# Autodesk Inventor assembly: WristRot
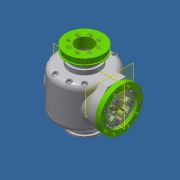
[picture p0: Inventor's stored thumbnail of the model, 180x180]
Saved by Autodesk Inventor 2016 (Build 200138000, 138)
## iProperties
Created: 2016-03-29
Part Number: WristRot
Material: Generisch
Document SubType Name: Assembly
Designer: 4ndreas
Mass: 560.727 g
Surface Area: 1571.35 cm^2
Volume: 276.943 cm^3
Density: 2.0247 g/cm^3
Parent: R5
Author: 4ndreas
## Documents named in this file (36)
- C:\Users\4ndreas\Documents\Inventor\betabots Mantis\Workspaces\Arbeitsbereich\v4\_assemblys\WristRot.iam
- C:\Users\4ndreas\Documents\Inventor\betabots Mantis\Workspaces\Arbeitsbereich\v4\_printed parts\WristRot_A.ipt
- C:\Users\4ndreas\Documents\Inventor\betabots Mantis\Workspaces\Arbeitsbereich\v4\_printed parts\WristRot_B.ipt
- C:\Users\4ndreas\Documents\Inventor\betabots Mantis\Workspaces\Arbeitsbereich\v4\_printed parts\WristRot_C.ipt
- C:\Users\4ndreas\Documents\Inventor\betabots Mantis\Workspaces\Arbeitsbereich\v4\_printed parts\WristRot_D.ipt
- C:\Users\4ndreas\Documents\Inventor\betabots Mantis\Workspaces\Arbeitsbereich\v4\_printed parts\WristRot_E.ipt
- C:\Users\4ndreas\Documents\Inventor\betabots Mantis\Workspaces\Arbeitsbereich\v4\_standard Parts\Distanzhuelse_M4x20mm.ipt
- C:\Users\4ndreas\Documents\Inventor\betabots Mantis\Libraries\Content Center Files\de-DE\DIN BEARING(1)\DIN 625 SKF - SKF 61807.ipt
- C:\Users\4ndreas\Documents\Inventor\betabots Mantis\Workspaces\Arbeitsbereich\v4\_Wrist_rev1\Wrist_rot_r1b\Konstruktions-Assistent\Stirnräder6.iam
- C:\Users\4ndreas\Documents\Inventor\betabots Mantis\Workspaces\Arbeitsbereich\v4\_standard Parts\Slipring_SNM012A-06.ipt
- C:\Users\4ndreas\Documents\Inventor\betabots Mantis\Libraries\Content Center Files\de-DE\DIN BEARING(1)\DIN 625 SKF - SKF 608.ipt
- C:\Users\4ndreas\Documents\Inventor\betabots Mantis\Workspaces\Arbeitsbereich\v4\_encoder\EncoderMagnet.ipt
- C:\Users\4ndreas\Documents\Inventor\betabots Mantis\Workspaces\Arbeitsbereich\v4\_Wrist_rev1\GripperRot.ipt
- C:\Users\4ndreas\Documents\Inventor\betabots Mantis\Libraries\Content Center Files\de-DE\DIN 125-1  A\DIN 125 - A 8,4.ipt
- C:\Users\4ndreas\Documents\Inventor\betabots Mantis\Workspaces\Arbeitsbereich\v4\_metal parts\SlipRingExtender.ipt
- C:\Users\4ndreas\Documents\Inventor\betabots Mantis\Libraries\Content Center Files\de-DE\DIN 985\DIN 985 - M6.ipt
- C:\Users\4ndreas\Documents\Inventor\betabots Mantis\Workspaces\Arbeitsbereich\v4\_Wrist_rev1\Wrist_rot_r1b\Konstruktions-Assistent\Stirnräder1.iam
- C:\Users\4ndreas\Documents\Inventor\betabots Mantis\Workspaces\Arbeitsbereich\v4\_Wrist_rev1\Wrist_rot_r1b\Konstruktions-Assistent\Welle1.iam
- C:\Users\4ndreas\Documents\Inventor\betabots Mantis\Workspaces\Arbeitsbereich\v4\_Wrist_rev1\Wrist_rot_r1b\Konstruktions-Assistent\Stirnräder3.iam
- C:\Users\4ndreas\Documents\Inventor\betabots Mantis\Workspaces\Arbeitsbereich\v4\_Wrist_rev1\Wrist_rot_r1b\Konstruktions-Assistent\Welle2.iam
- C:\Users\4ndreas\Documents\Inventor\betabots Mantis\Workspaces\Arbeitsbereich\v4\_motors\Stepper_42mm.ipt
- C:\Users\4ndreas\Documents\Inventor\betabots Mantis\Libraries\Content Center Files\de-DE\DIN 912\DIN 912 - M4 x 0,7 x 20 x 18,25.ipt
- C:\Users\4ndreas\Documents\Inventor\betabots Mantis\Libraries\Content Center Files\de-DE\DIN 7991(2)\DIN 7991 - M3x16.ipt
- C:\Users\4ndreas\Documents\Inventor\betabots Mantis\Workspaces\Arbeitsbereich\v4\_Wrist_rev1\RotGear_spacer.ipt
- C:\Users\4ndreas\Documents\Inventor\betabots Mantis\Workspaces\Arbeitsbereich\v4\_Wrist_rev1\Wrist_r1\Konstruktions-Assistent\Synchrone Riemenscheibe22.ipt
- C:\Users\4ndreas\Documents\Inventor\betabots Mantis\Libraries\Content Center Files\de-DE\DIN 7991(2)\DIN 7991 - M3x30.ipt
- C:\Users\4ndreas\Documents\Inventor\betabots Mantis\Workspaces\Arbeitsbereich\v4\_Wrist_rev1\RotGear_spacer_B.ipt
- C:\Users\4ndreas\Documents\Inventor\betabots Mantis\Workspaces\Arbeitsbereich\v4\_Wrist_rev1\WristMagnetMount.ipt
- C:\Users\4ndreas\Documents\Inventor\betabots Mantis\Libraries\Content Center Files\de-DE\DIN 7991(2)\DIN 7991 - M3x20.ipt
- C:\Users\4ndreas\Documents\Inventor\betabots Mantis\Workspaces\Arbeitsbereich\v4\_Wrist_rev1\GripperMountCover.ipt
- C:\Users\4ndreas\Documents\Inventor\betabots Mantis\Workspaces\Arbeitsbereich\v4\_encoder\encoderR1_mini.ipt
- C:\Users\4ndreas\Documents\Inventor\betabots Mantis\Libraries\Content Center Files\de-DE\DIN 625 SKF(4)\DIN 625 SKF - SKF 624-2Z.ipt
- C:\Users\4ndreas\Documents\Inventor\betabots Mantis\Libraries\Content Center Files\de-DE\DIN 125-1  A\DIN 125 - A 4,3.ipt
- C:\Users\4ndreas\Documents\Inventor\betabots Mantis\Libraries\Content Center Files\de-DE\DIN 912\DIN 912 - M3 x 0,5 x 8 x 6,75.ipt
- C:\Users\4ndreas\Documents\Inventor\betabots Mantis\Workspaces\Arbeitsbereich\v4\_encoder\encoder_neu.iam
- C:\Users\4ndreas\Documents\Inventor\betabots Mantis\Workspaces\Arbeitsbereich\v4\_Wrist_rev1\Wrist_EncoderMagnetMount.ipt
## Components (76 placed, 32 different names)
1. WristRot_A:1 — Fluchtend:1, Fluchtend:2, Fluchtend:3, Passend:1, Fluchtend:4, Passend:2, Passend:7, Passend:8, Passend:9, Passend:10, Passend:12, Passend:13, Passend:14, Passend:15, Passend:16, Passend:17, Passend:18, Passend:19, Passend:36, Passend:37, Passend:38, Passend:61, Passend:64, Passend:65, Einfügen:5, Einfügen:6, Einfügen:7, Einfügen:8, Einfügen:9, Passend:76, Passend:77, Passend:78, Passend:104, Winkel:1, Passend:115, Fluchtend:49
2. WristRot_B:1 — Passend:1, Fluchtend:4, Passend:2, Passend:3, Fluchtend:5, Passend:4, Passend:6, Fluchtend:48, Winkel:2
3. WristRot_C:1 — Passend:3, Fluchtend:5, Passend:4, Passend:5, Fluchtend:6, Passend:59
4. WristRot_D:1 — Passend:5, Passend:6, Fluchtend:6, Einfügen:1, Einfügen:2, Einfügen:3, Einfügen:4, Passend:11, Passend:79, Passend:80, Passend:81, Passend:82, Passend:83
5. WristRot_E:1 — Passend:7, Passend:8, Passend:66, Passend:67, Passend:68, Passend:69, Passend:70, Passend:71, Passend:72, Passend:73, Passend:74, Passend:75
6. Distanzhuelse_M4x20mm:1 — Passend:11, Fluchtend:7, Passend:19
7. Distanzhuelse_M4x20mm:2 — Passend:9, Fluchtend:8, Passend:17
8. Distanzhuelse_M4x20mm:3 — Passend:10, Fluchtend:7, Fluchtend:8, Fluchtend:9, Passend:18
9. Distanzhuelse_M4x20mm:4 — Passend:13, Fluchtend:10, Passend:14, Passend:15
10. Distanzhuelse_M4x20mm:5 — Passend:12, Fluchtend:9, Fluchtend:10, Passend:16
11. DIN 625 SKF SKF 61807:1 — Passend:38
12. Stirnräder:1 [sub-assembly] — Passend:45, Drehung:4
13. Slipring_SNM012A-06:1 — Passend:36, Winkel:2
14. DIN 625 SKF SKF 608:1 — Passend:35
15. EncoderMagnet:1 — Passend:109, Passend:110, Passend:118, Fluchtend:50
16. GripperRot:1 — Passend:34, Fluchtend:14, Passend:111, Passend:112, Passend:113, Passend:114
17. DIN 125-1 A A 8,4:1
18. SlipRingExtender:1 — Passend:34, Passend:35, Passend:37
19. DIN 985 - ersetzt durch DIN EN ISO 10511 M6:1
20. DIN 625 SKF- beidseitig abgedeckt SKF 624-2Z:2 — Fluchtend:48
21. DIN 625 SKF- beidseitig abgedeckt SKF 624-2Z:3
22. Stirnräder:2 [sub-assembly] — Passend:43, Passend:56, Drehung:3, Drehung:4
23. DIN 125-1 A A 4,3:1
24. Welle:1 [sub-assembly] — Passend:43, Passend:45
25. Stirnräder:3 [sub-assembly] — Passend:57, Passend:61, Passend:62, Passend:63, Drehung:3
26. DIN 625 SKF- beidseitig abgedeckt SKF 624-2Z:4
27. DIN 625 SKF- beidseitig abgedeckt SKF 624-2Z:1 — Passend:59
28. DIN 125-1 A A 4,3:2
29. Welle:2 [sub-assembly] — Passend:56, Passend:57
30. Stepper_42mm:1 — Passend:62, Passend:63, Passend:64, Passend:65
31. DIN 912 - ersetzt durch DIN EN ISO 4762 M4 x 20:1 — Einfügen:1
32. DIN 912 - ersetzt durch DIN EN ISO 4762 M4 x 20:2 — Einfügen:2
33. DIN 912 - ersetzt durch DIN EN ISO 4762 M4 x 20:3 — Einfügen:3
34. DIN 912 - ersetzt durch DIN EN ISO 4762 M4 x 20:4 — Einfügen:4
35. DIN 912 - ersetzt durch DIN EN ISO 4762 M4 x 20:5 — Einfügen:5
36. DIN 912 - ersetzt durch DIN EN ISO 4762 M4 x 20:6 — Einfügen:6
37. DIN 912 - ersetzt durch DIN EN ISO 4762 M4 x 20:7 — Einfügen:7
38. DIN 912 - ersetzt durch DIN EN ISO 4762 M4 x 20:8 — Einfügen:8
39. DIN 912 - ersetzt durch DIN EN ISO 4762 M4 x 20:9 — Einfügen:9
40. DIN 7991 M3x16:1 — Passend:66
41. DIN 7991 M3x16:2 — Passend:67
42. DIN 7991 M3x16:3 — Passend:68
43. DIN 7991 M3x16:4 — Passend:69
44. DIN 7991 M3x16:5 — Passend:70
45. DIN 7991 M3x16:6 — Passend:71, Passend:104
46. DIN 7991 M3x16:7 — Passend:72
47. DIN 7991 M3x16:8 — Passend:73
48. DIN 7991 M3x16:9 — Passend:74
49. DIN 7991 M3x16:10 — Passend:75
50. RotGear_spacer:1 — Passend:76, Passend:77, Passend:78, Passend:84, Passend:85, Passend:86
51. RotGear_spacer_B:1 — Passend:79, Passend:80, Passend:81, Fluchtend:13
52. DIN 912 - ersetzt durch DIN EN ISO 4762 M4 x 20:10 — Passend:82, Passend:83
53. Synchrone Riemenscheibe2:1 — Passend:84, Passend:85, Passend:86, Passend:87, Passend:88, Passend:89, Passend:90, Passend:91, Passend:92, Passend:93, Passend:94, Passend:116
54. DIN 7991 M3x30:1 — Passend:87
55. DIN 7991 M3x30:2 — Passend:88
56. DIN 7991 M3x30:3 — Passend:89
57. DIN 7991 M3x30:4 — Passend:90
58. DIN 7991 M3x30:5 — Passend:91
59. DIN 7991 M3x30:6 — Passend:92
60. DIN 7991 M3x30:7 — Passend:93
61. DIN 7991 M3x30:8 — Passend:94
62. WristMagnetMount:1 — Fluchtend:13, Passend:95, Passend:96, Passend:99, Passend:101, Passend:117
63. DIN 7991 M3x20:1 — Passend:95
64. DIN 7991 M3x20:2 — Passend:96
65. DIN 7991 M3x20:5 — Passend:99
66. DIN 7991 M3x20:7 — Passend:101
67. EncoderMagnet:2 — Passend:117
68. GripperMountCover:1 — Fluchtend:14, Passend:105, Passend:106, Passend:107
69. DIN 7991 M3x16:11 — Passend:105
70. DIN 7991 M3x16:12 — Passend:106
71. DIN 7991 M3x16:13 — Passend:107
72. encoderR1_mini:1 — Passend:109, Passend:110, Winkel:1
73. DIN 912 - ersetzt durch DIN EN ISO 4762 M3 x 8:1 — Passend:111, Passend:112
74. DIN 912 - ersetzt durch DIN EN ISO 4762 M3 x 8:2 — Passend:113, Passend:114
75. encoder_neu:1 [sub-assembly] — Passend:115, Fluchtend:49, Passend:116
76. Wrist_EncoderMagnetMount:1 — Passend:118, Fluchtend:50
## Relationships (140: Mate 109, Flush 16, Insert 9, RelateRotation 4, Angle 2)
- Fluchtend:1 [Flush]: WristRot_A:1
- Fluchtend:2 [Flush]: WristRot_A:1
- Fluchtend:3 [Flush]: WristRot_A:1
- Passend:1 [Mate]: WristRot_A:1 ↔ WristRot_B:1
- Fluchtend:4 [Flush]: WristRot_A:1 ↔ WristRot_B:1
- Passend:2 [Mate]: WristRot_A:1 ↔ WristRot_B:1
- Passend:3 [Mate]: WristRot_B:1 ↔ WristRot_C:1
- Fluchtend:5 [Flush]: WristRot_B:1 ↔ WristRot_C:1
- Passend:4 [Mate]: WristRot_B:1 ↔ WristRot_C:1
- Passend:5 [Mate]: WristRot_C:1 ↔ WristRot_D:1
- Passend:6 [Mate]: WristRot_B:1 ↔ WristRot_D:1
- Fluchtend:6 [Flush]: WristRot_C:1 ↔ WristRot_D:1
- Passend:7 [Mate]: WristRot_A:1 ↔ WristRot_E:1
- Passend:8 [Mate]: WristRot_A:1 ↔ WristRot_E:1
- Passend:9 [Mate]: WristRot_A:1 ↔ Distanzhuelse_M4x20mm:2
- Passend:10 [Mate]: WristRot_A:1 ↔ Distanzhuelse_M4x20mm:3
- Passend:11 [Mate]: WristRot_D:1 ↔ Distanzhuelse_M4x20mm:1
- Fluchtend:7 [Flush]: Distanzhuelse_M4x20mm:1 ↔ Distanzhuelse_M4x20mm:3
- Fluchtend:8 [Flush]: Distanzhuelse_M4x20mm:2 ↔ Distanzhuelse_M4x20mm:3
- Passend:12 [Mate]: WristRot_A:1 ↔ Distanzhuelse_M4x20mm:5
- Passend:13 [Mate]: WristRot_A:1 ↔ Distanzhuelse_M4x20mm:4
- Fluchtend:9 [Flush]: Distanzhuelse_M4x20mm:3 ↔ Distanzhuelse_M4x20mm:5
- Fluchtend:10 [Flush]: Distanzhuelse_M4x20mm:4 ↔ Distanzhuelse_M4x20mm:5
- Passend:14 [Mate]: WristRot_A:1 ↔ Distanzhuelse_M4x20mm:4
- Passend:15 [Mate]: WristRot_A:1 ↔ Distanzhuelse_M4x20mm:4
- Passend:16 [Mate]: WristRot_A:1 ↔ Distanzhuelse_M4x20mm:5
- Passend:17 [Mate]: WristRot_A:1 ↔ Distanzhuelse_M4x20mm:2
- Passend:18 [Mate]: WristRot_A:1 ↔ Distanzhuelse_M4x20mm:3
- Passend:19 [Mate]: WristRot_A:1 ↔ Distanzhuelse_M4x20mm:1
- [Mate]: Slipring_SNM012A-06:1 ↔ DIN 625 SKF SKF 608:1
- [Mate]: Slipring_SNM012A-06:1 ↔ EncoderMagnet:1
- [Mate] (3 mm): Slipring_SNM012A-06:1 ↔ EncoderMagnet:1
- [Mate]: DIN 625 SKF SKF 61807:1 ↔ GripperRot:1
- [Mate]: DIN 625 SKF SKF 61807:1 ↔ GripperRot:1
- [Mate]: Stirnräder:1 ↔ DIN 125-1 A A 8,4:1
- [Mate]: DIN 625 SKF SKF 608:1 ↔ DIN 125-1 A A 8,4:1
- [Mate]: Stirnräder:1 ↔ DIN 125-1 A A 8,4:1
- [Mate]: Stirnräder:1 ↔ SlipRingExtender:1
- [Mate]: Stirnräder:1 ↔ SlipRingExtender:1
- [Mate]: SlipRingExtender:1 ↔ DIN 985 - ersetzt durch DIN EN ISO 10511 M6:1
- [Mate]: Stirnräder:1 ↔ DIN 985 - ersetzt durch DIN EN ISO 10511 M6:1
- [Mate]: Stirnräder:1 ↔ GripperRot:1
- [Mate]: Stirnräder:1 ↔ GripperRot:1
- [RelateRotation] (1 ul): SlipRingExtender:1 ↔ DIN 985 - ersetzt durch DIN EN ISO 10511 M6:1
- [RelateRotation] (1 ul): Stirnräder:1 ↔ DIN 985 - ersetzt durch DIN EN ISO 10511 M6:1
- Passend:34 [Mate]: GripperRot:1 ↔ SlipRingExtender:1
- Passend:35 [Mate]: DIN 625 SKF SKF 608:1 ↔ SlipRingExtender:1
- Passend:36 [Mate]: WristRot_A:1 ↔ Slipring_SNM012A-06:1
- Passend:37 [Mate]: WristRot_A:1 ↔ SlipRingExtender:1
- Passend:38 [Mate]: WristRot_A:1 ↔ DIN 625 SKF SKF 61807:1
- [Mate]: DIN 625 SKF- beidseitig abgedeckt SKF 624-2Z:3 ↔ DIN 125-1 A A 4,3:1
- [Mate]: Stirnräder:2 ↔ DIN 125-1 A A 4,3:1
- [Mate]: DIN 625 SKF- beidseitig abgedeckt SKF 624-2Z:3 ↔ DIN 125-1 A A 4,3:1
- [Mate]: DIN 625 SKF- beidseitig abgedeckt SKF 624-2Z:2 ↔ Welle:1
- Passend:43 [Mate]: Stirnräder:2 ↔ Welle:1
- [Mate]: DIN 625 SKF- beidseitig abgedeckt SKF 624-2Z:3 ↔ Welle:1
- Passend:45 [Mate]: Stirnräder:1 ↔ Welle:1
- [Mate]: WristRot_B:1 ↔ DIN 625 SKF- beidseitig abgedeckt SKF 624-2Z:2
- Fluchtend:48 [Flush]: WristRot_B:1 ↔ DIN 625 SKF- beidseitig abgedeckt SKF 624-2Z:2
- [Mate]: WristRot_B:1 ↔ DIN 625 SKF- beidseitig abgedeckt SKF 624-2Z:3
- [Mate]: Stirnräder:3 ↔ DIN 625 SKF- beidseitig abgedeckt SKF 624-2Z:4
- [Mate] (0.5 mm): Stirnräder:3 ↔ DIN 625 SKF- beidseitig abgedeckt SKF 624-2Z:4
- [Mate]: DIN 625 SKF- beidseitig abgedeckt SKF 624-2Z:1 ↔ DIN 125-1 A A 4,3:2
- [Mate]: DIN 625 SKF- beidseitig abgedeckt SKF 624-2Z:4 ↔ DIN 125-1 A A 4,3:2
- [Mate]: DIN 625 SKF- beidseitig abgedeckt SKF 624-2Z:1 ↔ Welle:2
- [Flush] (-1 mm): Stirnräder:3 ↔ Welle:2
- Passend:56 [Mate]: Stirnräder:2 ↔ Welle:2
- Passend:57 [Mate]: Stirnräder:3 ↔ Welle:2
- [Mate]: WristRot_C:1 ↔ DIN 625 SKF- beidseitig abgedeckt SKF 624-2Z:1
- Passend:59 [Mate]: WristRot_C:1 ↔ DIN 625 SKF- beidseitig abgedeckt SKF 624-2Z:1
- [Mate]: Stirnräder:2 ↔ DIN 125-1 A A 4,3:2
- Passend:61 [Mate]: WristRot_A:1 ↔ Stirnräder:3
- Passend:62 [Mate]: Stirnräder:3 ↔ Stepper_42mm:1
- Passend:63 [Mate]: Stirnräder:3 ↔ Stepper_42mm:1
- Passend:64 [Mate]: WristRot_A:1 ↔ Stepper_42mm:1
- Passend:65 [Mate]: WristRot_A:1 ↔ Stepper_42mm:1
- Einfügen:1 [Insert]: WristRot_D:1 ↔ DIN 912 - ersetzt durch DIN EN ISO 4762 M4 x 20:1
- Einfügen:2 [Insert]: WristRot_D:1 ↔ DIN 912 - ersetzt durch DIN EN ISO 4762 M4 x 20:2
- Einfügen:3 [Insert]: WristRot_D:1 ↔ DIN 912 - ersetzt durch DIN EN ISO 4762 M4 x 20:3
- Einfügen:4 [Insert]: WristRot_D:1 ↔ DIN 912 - ersetzt durch DIN EN ISO 4762 M4 x 20:4
- Einfügen:5 [Insert]: WristRot_A:1 ↔ DIN 912 - ersetzt durch DIN EN ISO 4762 M4 x 20:5
- Einfügen:6 [Insert]: WristRot_A:1 ↔ DIN 912 - ersetzt durch DIN EN ISO 4762 M4 x 20:6
- Einfügen:7 [Insert]: WristRot_A:1 ↔ DIN 912 - ersetzt durch DIN EN ISO 4762 M4 x 20:7
- Einfügen:8 [Insert]: WristRot_A:1 ↔ DIN 912 - ersetzt durch DIN EN ISO 4762 M4 x 20:8
- Einfügen:9 [Insert]: WristRot_A:1 ↔ DIN 912 - ersetzt durch DIN EN ISO 4762 M4 x 20:9
- Passend:66 [Mate]: WristRot_E:1 ↔ DIN 7991 M3x16:1
- Passend:67 [Mate]: WristRot_E:1 ↔ DIN 7991 M3x16:2
- Passend:68 [Mate]: WristRot_E:1 ↔ DIN 7991 M3x16:3
- Passend:69 [Mate]: WristRot_E:1 ↔ DIN 7991 M3x16:4
- Passend:70 [Mate]: WristRot_E:1 ↔ DIN 7991 M3x16:5
- Passend:71 [Mate]: WristRot_E:1 ↔ DIN 7991 M3x16:6
- Passend:72 [Mate]: WristRot_E:1 ↔ DIN 7991 M3x16:7
- Passend:73 [Mate]: WristRot_E:1 ↔ DIN 7991 M3x16:8
- Passend:74 [Mate]: WristRot_E:1 ↔ DIN 7991 M3x16:9
- Passend:75 [Mate]: WristRot_E:1 ↔ DIN 7991 M3x16:10
- Passend:76 [Mate]: WristRot_A:1 ↔ RotGear_spacer:1
- Passend:77 [Mate]: WristRot_A:1 ↔ RotGear_spacer:1
- Passend:78 [Mate]: WristRot_A:1 ↔ RotGear_spacer:1
- Passend:79 [Mate]: WristRot_D:1 ↔ RotGear_spacer_B:1
- Passend:80 [Mate]: WristRot_D:1 ↔ RotGear_spacer_B:1
- Passend:81 [Mate]: WristRot_D:1 ↔ RotGear_spacer_B:1
- Passend:82 [Mate]: WristRot_D:1 ↔ DIN 912 - ersetzt durch DIN EN ISO 4762 M4 x 20:10
- Passend:83 [Mate]: WristRot_D:1 ↔ DIN 912 - ersetzt durch DIN EN ISO 4762 M4 x 20:10
- Passend:84 [Mate]: RotGear_spacer:1 ↔ Synchrone Riemenscheibe2:1
- Passend:85 [Mate]: RotGear_spacer:1 ↔ Synchrone Riemenscheibe2:1
- Passend:86 [Mate]: RotGear_spacer:1 ↔ Synchrone Riemenscheibe2:1
- Passend:87 [Mate]: Synchrone Riemenscheibe2:1 ↔ DIN 7991 M3x30:1
- Passend:88 [Mate]: Synchrone Riemenscheibe2:1 ↔ DIN 7991 M3x30:2
- Passend:89 [Mate]: Synchrone Riemenscheibe2:1 ↔ DIN 7991 M3x30:3
- Passend:90 [Mate]: Synchrone Riemenscheibe2:1 ↔ DIN 7991 M3x30:4
- Passend:91 [Mate]: Synchrone Riemenscheibe2:1 ↔ DIN 7991 M3x30:5
- Passend:92 [Mate]: Synchrone Riemenscheibe2:1 ↔ DIN 7991 M3x30:6
- Passend:93 [Mate]: Synchrone Riemenscheibe2:1 ↔ DIN 7991 M3x30:7
- Passend:94 [Mate]: Synchrone Riemenscheibe2:1 ↔ DIN 7991 M3x30:8
- Fluchtend:13 [Flush] (-3.5 mm): RotGear_spacer_B:1 ↔ WristMagnetMount:1
- Passend:95 [Mate]: WristMagnetMount:1 ↔ DIN 7991 M3x20:1
- Passend:96 [Mate]: WristMagnetMount:1 ↔ DIN 7991 M3x20:2
- Passend:99 [Mate]: WristMagnetMount:1 ↔ DIN 7991 M3x20:5
- Passend:101 [Mate]: WristMagnetMount:1 ↔ DIN 7991 M3x20:7
- Passend:104 [Mate]: WristRot_A:1 ↔ DIN 7991 M3x16:6
- Fluchtend:14 [Flush]: GripperRot:1 ↔ GripperMountCover:1
- Passend:105 [Mate]: GripperMountCover:1 ↔ DIN 7991 M3x16:11
- Passend:106 [Mate]: GripperMountCover:1 ↔ DIN 7991 M3x16:12
- Passend:107 [Mate]: GripperMountCover:1 ↔ DIN 7991 M3x16:13
- Passend:109 [Mate]: EncoderMagnet:1 ↔ encoderR1_mini:1
- Passend:110 [Mate] (0.5 mm): EncoderMagnet:1 ↔ encoderR1_mini:1
- Winkel:1 [Angle] (0 deg): WristRot_A:1 ↔ encoderR1_mini:1
- Winkel:2 [Angle] (0 deg): WristRot_B:1 ↔ Slipring_SNM012A-06:1
- Drehung:3 [RelateRotation] (1.333 ul): Stirnräder:2 ↔ Stirnräder:3
- Drehung:4 [RelateRotation] (1.333 ul): Stirnräder:1 ↔ Stirnräder:2
- Passend:111 [Mate]: GripperRot:1 ↔ DIN 912 - ersetzt durch DIN EN ISO 4762 M3 x 8:1
- Passend:112 [Mate]: GripperRot:1 ↔ DIN 912 - ersetzt durch DIN EN ISO 4762 M3 x 8:1
- Passend:113 [Mate]: GripperRot:1 ↔ DIN 912 - ersetzt durch DIN EN ISO 4762 M3 x 8:2
- Passend:114 [Mate]: GripperRot:1 ↔ DIN 912 - ersetzt durch DIN EN ISO 4762 M3 x 8:2
- Passend:115 [Mate]: WristRot_A:1 ↔ encoder_neu:1
- Fluchtend:49 [Flush]: WristRot_A:1 ↔ encoder_neu:1
- Passend:116 [Mate]: Synchrone Riemenscheibe2:1 ↔ encoder_neu:1
- Passend:117 [Mate]: WristMagnetMount:1 ↔ EncoderMagnet:2
- Passend:118 [Mate]: EncoderMagnet:1 ↔ Wrist_EncoderMagnetMount:1
- Fluchtend:50 [Flush]: EncoderMagnet:1 ↔ Wrist_EncoderMagnetMount:1
